# Autodesk Inventor assembly: RUKA ROBOT ASSEMBLY
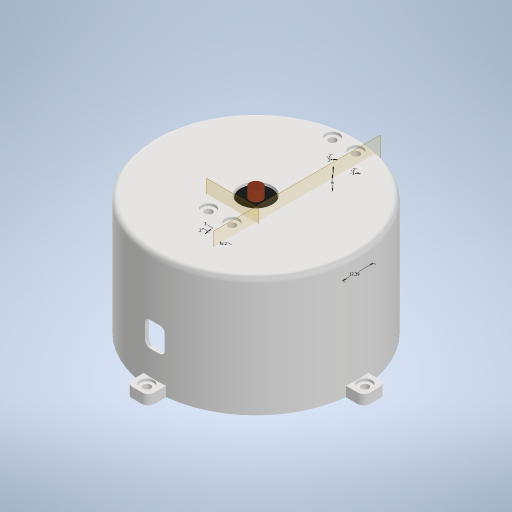
[picture p0: Inventor's stored thumbnail of the model, 512x512]
Saved by Autodesk Inventor 2023 (Build 270158000, 158)
## iProperties
Created: 2025-04-11
Part Number: RUKA ROBOT ASSEMBLY
Document SubType Name: Assembly
Designer: janpa
Author: janpa
## Documents named in this file (3)
- C:\Users\janpa\OneDrive\Plocha\Hackaton\Hackathon25\3d\RUKA ROBOT ASSEMBLY.iam
- C:\Users\janpa\Downloads\MG995-Servo.ipt
- C:\Users\janpa\OneDrive\Plocha\Hackaton\Hackathon25\3d\ruka base.ipt
## Components (2 placed, 2 different names)
1. MG995-Servo:1 — Mate:1
2. ruka base:1 — Mate:1
## Relationships (1: Mate 1)
- Mate:1: MG995-Servo:1 ↔ ruka base:1
